# Autodesk Inventor assembly: Assembly1
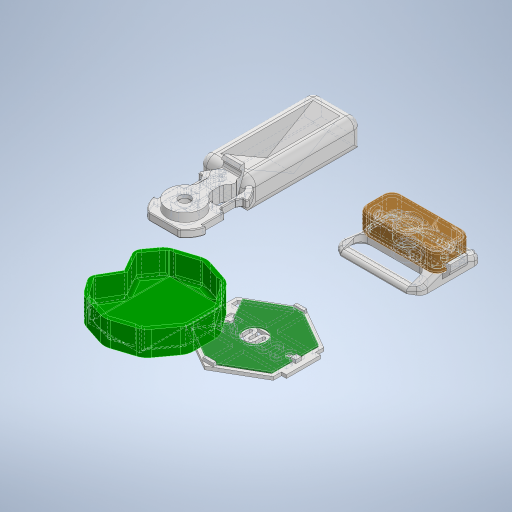
[picture p0: Inventor's stored thumbnail of the model, 512x512]
Saved by Autodesk Inventor 2024 (Build 280153000, 153)
## iProperties
Created: 2022-10-19
Part Number: Assembly1
Document SubType Name: Assembly
Designer: jevan
Author: jevan
## Documents named in this file (24)
- C:\Users\jevan\Documents\GitHub\LilypadVR\V4\CAD\Models\Assembly1.iam
- C:\Users\jevan\Documents\GitHub\LilypadVR\V4\CAD\Models\PCB.ipt
- C:\Users\jevan\Documents\GitHub\LilypadVR\V4\CAD\Models\PJ-242.ipt
- C:\Users\jevan\Documents\Models\tp4056-charging-module-type-c-1.snapshot.1\TP4056_Charging_Module_Type_C.ipt
- C:\Users\jevan\Documents\GitHub\LilypadVR\V4\CAD\Models\LilypadShellProto1.ipt
- C:\Users\jevan\Documents\GitHub\LilypadVR\V4\CAD\Models\ChargeLED.ipt
- C:\Users\jevan\Documents\GitHub\LilypadVR\V4\CAD\Models\ESPLED.ipt
- C:\Users\jevan\Documents\GitHub\LilypadVR\V4\CAD\Models\Battery.ipt
- C:\Users\jevan\Documents\GitHub\LilypadVR\V4\CAD\Models\PCBAux.ipt
- C:\Users\jevan\Documents\GitHub\LilypadVR\V4\CAD\Models\AUXShell.ipt
- C:\Users\jevan\Documents\GitHub\LilypadVR\V4\CAD\Models\SKRTLA.ipt
- C:\Users\jevan\Documents\GitHub\LilypadVR\V4\CAD\Models\AUXShellLid.ipt
- C:\Users\jevan\Documents\GitHub\LilypadVR\V4\CAD\Models\ShellLid.ipt
- C:\Users\jevan\Documents\GitHub\LilypadVR\V4\CAD\Models\CalibrationBlock.ipt
- C:\Users\jevan\Documents\GitHub\LilypadVR\V4\CAD\Models\ButtonInsert.ipt
- C:\Users\jevan\Documents\GitHub\LilypadVR\V4\CAD\Models\AccessoryScrew.ipt
- C:\Users\jevan\Documents\GitHub\LilypadVR\V4\CAD\Models\LilypadClip.ipt
- C:\Users\jevan\Documents\GitHub\LilypadVR\V4\CAD\Models\ShellFix.ipt
- C:\Users\jevan\Documents\GitHub\LilypadVR\V4\CAD\Models\LightPipe.ipt
- C:\Users\jevan\Documents\GitHub\LilypadVR\V5\CAD\Models\ShellMockup_01.ipt
- C:\Users\jevan\Documents\GitHub\LilypadVR\V4\CAD\Models\CalibrationPlate.ipt
- C:\Users\jevan\Documents\GitHub\LilypadVR\V4\CAD\Models\LilypadClipNew.ipt
- C:\Users\jevan\Documents\GitHub\LilypadVR\V4\CAD\Models\PrototypeModels\GoProAdapter.ipt
- C:\Users\jevan\Documents\GitHub\LilypadVR\V4\CAD\Models\PrototypeModels\BareCalibrationClip.ipt
## Components (27 placed, 23 different names)
1. PCB:1 — Flush:1, Mate:1, Flush:3, Flush:6, Mate:4, Mate:5, Flush:8, Flush:9, Flush:11, Mate:15, Mate:16, Flush:20, Flush:21, Mate:17, Flush:22, Flush:23, Flush:25, Mate:35, Mate:37, Angle:1, Flush:35, Mate:53, Mate:54
2. PJ-242:1 — Flush:1, Flush:30
3. TP4056_Charging_Module_Type_C:1 — Mate:1, Flush:3, Flush:6
4. LilypadShellProto1:1 — Mate:4, Mate:5
5. ChargeLED:1 — Flush:8, Flush:25, Mate:22
6. ESPLED:1 — Flush:9, Flush:11, Mate:15, Mate:22
7. Battery:1 — Mate:23, Mate:24, Mate:25
8. PCBAux:1 — Flush:12, Mate:11, Flush:13, Flush:24, Mate:18
9. PJ-242:2 — Flush:12, Mate:11, Flush:24
10. AUXShell:1 — Flush:13, Mate:18, Flush:26, Mate:33, Flush:31, Mate:42, Mate:46, Insert:1
11. SKRTLA:1 — Mate:17, Flush:22, Flush:23
12. SKRTLA:2 — Mate:16, Flush:20, Flush:21
13. AUXShellLid:1 — Flush:26, Flush:31, Mate:42
14. ShellLid:1 — Mate:23, Mate:24, Mate:25, Mate:34, Flush:27, Flush:30, Flush:34, Mate:51
15. CalibrationBlock:1 — Mate:45, Mate:47
16. ButtonInsert:1 — Flush:29
17. AccessoryScrew:1 — Mate:34, Mate:38, Mate:40
18. AccessoryScrew:2 — Mate:33, Flush:32
19. LilypadClip:1 — Mate:39, Mate:40
20. ShellFix:1 — Flush:27, Mate:35, Mate:37, Mate:38, Mate:39, Flush:29, Mate:45, Mate:47, Flush:33, Mate:48, Mate:49, Mate:50, Angle:1, Flush:34, Mate:51, Mate:52
21. LilypadClip:2 — Mate:46, Insert:1, Flush:32
22. LightPipe:1 — Flush:33, Mate:48, Mate:49
23. ShellMockup_01:1
24. CalibrationPlate:1
25. LilypadClipNew:1 — Mate:50, Mate:52
26. GoProAdapter:1
27. BareCalibrationClip:1 — Flush:35, Mate:53, Mate:54
## Relationships (55: Mate 30, Flush 23, Insert 1, Angle 1)
- Flush:1: PCB:1 ↔ PJ-242:1
- Mate:1: PCB:1 ↔ TP4056_Charging_Module_Type_C:1
- Flush:3: PCB:1 ↔ TP4056_Charging_Module_Type_C:1
- Flush:6 (1.7 mm): PCB:1 ↔ TP4056_Charging_Module_Type_C:1
- Mate:4: PCB:1 ↔ LilypadShellProto1:1
- Mate:5: PCB:1 ↔ LilypadShellProto1:1
- Flush:8: PCB:1 ↔ ChargeLED:1
- Flush:9: PCB:1 ↔ ESPLED:1
- Flush:11: PCB:1 ↔ ESPLED:1
- Flush:12: PCBAux:1 ↔ PJ-242:2
- Mate:11: PCBAux:1 ↔ PJ-242:2
- Flush:13: PCBAux:1 ↔ AUXShell:1
- Mate:15 (7.85 mm): PCB:1 ↔ ESPLED:1
- Mate:16: PCB:1 ↔ SKRTLA:2
- Flush:20 (0.46 mm): PCB:1 ↔ SKRTLA:2
- Flush:21: PCB:1 ↔ SKRTLA:2
- Mate:17: PCB:1 ↔ SKRTLA:1
- Flush:22: PCB:1 ↔ SKRTLA:1
- Flush:23 (16.67 mm): PCB:1 ↔ SKRTLA:1
- Flush:24 (5.5 mm): PCBAux:1 ↔ PJ-242:2
- Mate:18: PCBAux:1 ↔ AUXShell:1
- Flush:25 (1.1 mm): PCB:1 ↔ ChargeLED:1
- Mate:22 (2.2 mm): ChargeLED:1 ↔ ESPLED:1
- Mate:23: Battery:1 ↔ ShellLid:1
- Mate:24 (1 mm): Battery:1 ↔ ShellLid:1
- Mate:25: Battery:1 ↔ ShellLid:1
- Flush:26: AUXShell:1 ↔ AUXShellLid:1
- Mate:33: AUXShell:1 ↔ AccessoryScrew:2
- Mate:34 (0.5 mm): ShellLid:1 ↔ AccessoryScrew:1
- Flush:27: ShellLid:1 ↔ ShellFix:1
- Mate:35: PCB:1 ↔ ShellFix:1
- Mate:37: PCB:1 ↔ ShellFix:1
- Mate:38: AccessoryScrew:1 ↔ ShellFix:1
- Mate:39: LilypadClip:1 ↔ ShellFix:1
- Mate:40: AccessoryScrew:1 ↔ LilypadClip:1
- Flush:29 (-2 mm): ButtonInsert:1 ↔ ShellFix:1
- Flush:30: PJ-242:1 ↔ ShellLid:1
- Flush:31: AUXShell:1 ↔ AUXShellLid:1
- Mate:42: AUXShell:1 ↔ AUXShellLid:1
- Mate:45: CalibrationBlock:1 ↔ ShellFix:1
- Mate:46: AUXShell:1 ↔ LilypadClip:2
- Insert:1: AUXShell:1 ↔ LilypadClip:2
- Flush:32: AccessoryScrew:2 ↔ LilypadClip:2
- Mate:47: CalibrationBlock:1 ↔ ShellFix:1
- Flush:33: ShellFix:1 ↔ LightPipe:1
- Mate:48 (0.1 mm): ShellFix:1 ↔ LightPipe:1
- Mate:49: ShellFix:1 ↔ LightPipe:1
- Mate:50: ShellFix:1 ↔ LilypadClipNew:1
- Angle:1 (0 deg): PCB:1 ↔ ShellFix:1
- Flush:34: ShellLid:1 ↔ ShellFix:1
- Mate:51: ShellLid:1 ↔ ShellFix:1
- Mate:52: ShellFix:1 ↔ LilypadClipNew:1
- Flush:35: PCB:1 ↔ BareCalibrationClip:1
- Mate:53: PCB:1 ↔ BareCalibrationClip:1
- Mate:54 (0.2 mm): PCB:1 ↔ BareCalibrationClip:1
